# Autodesk Inventor assembly: Design 1
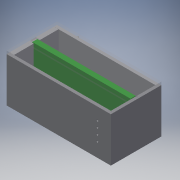
[picture p0: Inventor's stored thumbnail of the model, 180x180]
Saved by Autodesk Inventor 2018.3 (Build 223284000, 284)
## iProperties
Created: 2020-11-10
Part Number: Design 1
Document SubType Name: Assembly
Designer: daanv
Author: daanv
## Documents named in this file (8)
- C:\Users\daanv\OneDrive\Documenten\Life\New folder\Design 1.iam
- C:\Users\daanv\OneDrive\Documenten\Life\New folder\Achterplaat.ipt
- C:\Users\daanv\OneDrive\Documenten\Life\New folder\Voorplaat.ipt
- C:\Users\daanv\OneDrive\Documenten\Life\New folder\Zijplaat 1.ipt
- C:\Users\daanv\OneDrive\Documenten\Life\New folder\Zijplaat 3.ipt
- C:\Users\daanv\OneDrive\Documenten\Life\New folder\Zijplaat 4.ipt
- C:\Users\daanv\OneDrive\Documenten\Life\New folder\Token module.ipt
- C:\Users\daanv\OneDrive\Documenten\Life\New folder\Zijplaat 2.ipt
## Components (7 placed, 7 different names)
1. Achterplaat:1 — Mate:1, Mate:2, Mate:4
2. Voorplaat:1 — Mate:7, Mate:8, Mate:10, Mate:11, Mate:14, Mate:16
3. Zijplaat 1:1 — Mate:1, Mate:2, Mate:3, Mate:5, Mate:7, Mate:9, Mate:13
4. Zijplaat 3:1 — Mate:9, Mate:10, Mate:11
5. Zijplaat 4:1 — Mate:3, Mate:4, Mate:5, Mate:8, Mate:15
6. Token module:1 — Mate:13, Mate:14
7. Zijplaat 2:1 — Mate:15, Mate:16
## Relationships (14: Mate 14)
- Mate:1: Achterplaat:1 ↔ Zijplaat 1:1
- Mate:2: Achterplaat:1 ↔ Zijplaat 1:1
- Mate:3: Zijplaat 1:1 ↔ Zijplaat 4:1
- Mate:4: Achterplaat:1 ↔ Zijplaat 4:1
- Mate:5: Zijplaat 1:1 ↔ Zijplaat 4:1
- Mate:7: Voorplaat:1 ↔ Zijplaat 1:1
- Mate:8: Voorplaat:1 ↔ Zijplaat 4:1
- Mate:9: Zijplaat 1:1 ↔ Zijplaat 3:1
- Mate:10: Voorplaat:1 ↔ Zijplaat 3:1
- Mate:11: Voorplaat:1 ↔ Zijplaat 3:1
- Mate:13: Zijplaat 1:1 ↔ Token module:1
- Mate:14: Voorplaat:1 ↔ Token module:1
- Mate:15: Zijplaat 4:1 ↔ Zijplaat 2:1
- Mate:16: Voorplaat:1 ↔ Zijplaat 2:1
